# Autodesk Inventor assembly: Assembly2
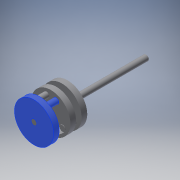
[picture p0: Inventor's stored thumbnail of the model, 180x180]
Saved by Autodesk Inventor 2017 (Build 210142000, 142)
## iProperties
Created: 2021-05-19
Part Number: Assembly2
Document SubType Name: Assembly
Designer: majch
Author: majch
## Documents named in this file (6)
- E:\inventor\mocowanie\Assembly2.iam
- E:\inventor\mocowanie\ogolny_walek-011.ipt
- E:\inventor\mocowanie\ogolny_walek.ipt
- E:\inventor\mocowanie\test1.ipt
- E:\inventor\mocowanie\Part6-01.ipt
- E:\inventor\mocowanie\test2.ipt
## Components (4 placed, 3 different names)
1. ogolny_walek-011:1 — Mate:2, Mate:3, Mate:4, Flush:3
2. test1:2 — Mate:2, Flush:2
3. Part6-01:1 — Mate:3, Flush:2, Mate:5
4. test1:3 — Mate:4, Flush:3, Mate:5
## Relationships (6: Mate 4, Flush 2)
- Mate:2: ogolny_walek-011:1 ↔ test1:2
- Mate:3: ogolny_walek-011:1 ↔ Part6-01:1
- Flush:2: test1:2 ↔ Part6-01:1
- Mate:4: ogolny_walek-011:1 ↔ test1:3
- Flush:3: ogolny_walek-011:1 ↔ test1:3
- Mate:5: Part6-01:1 ↔ test1:3
